# Autodesk Inventor assembly: projectorPanTiltSystem02
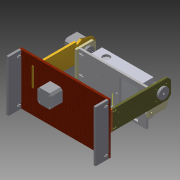
[picture p0: Inventor's stored thumbnail of the model, 180x180]
Saved by Autodesk Inventor 2013 (Build 170138000, 138)
## iProperties
Created: 2014-06-13
Part Number: projectorPanTiltSystem02
Document SubType Name: Assembly
Designer: Byron
Author: Byron
## Documents named in this file (15)
- C:\Users\Nano\Documents\InventorByron\InventorMasterProject\projectorPanTilt02-2014-06-23\projectorPanTilt02\projectorPanTiltSystem02.iam
- C:\Users\Nano\Documents\InventorByron\InventorMasterProject\projectorPanTilt-2014-06-23\projectorPanTilt\stepper42BYGH007.ipt
- C:\Users\Nano\Documents\InventorByron\InventorMasterProject\projectorPanTilt-2014-06-23\projectorPanTilt\aaxaProjector01.ipt
- C:\Users\Nano\Documents\InventorByron\InventorMasterProject\projectorPanTilt02-2014-06-23\projectorPanTilt02\projectorMountingBase.ipt
- C:\Users\Nano\Documents\InventorByron\InventorMasterProject\projectorPanTilt02-2014-06-23\projectorPanTilt02\projectorMountSide.ipt
- C:\Users\Nano\Documents\InventorByron\InventorMasterProject\projectorPanTilt02-2014-06-23\projectorPanTilt02\tiltColumnStepperSide02.ipt
- C:\Users\Nano\Documents\InventorByron\InventorMasterProject\projectorPanTilt02-2014-06-23\projectorPanTilt02\stepperShaftCollar.ipt
- C:\Users\Nano\Documents\InventorByron\InventorMasterProject\projectorPanTilt02-2014-06-23\projectorPanTilt02\tiltStructureCrossBeam.ipt
- C:\Users\Nano\Documents\InventorByron\InventorMasterProject\projectorPanTilt02-2014-06-23\projectorPanTilt02\tiltColumnNonStepperSide02.ipt
- C:\Users\Nano\Documents\InventorByron\InventorMasterProject\projectorPanTilt02-2014-06-23\projectorPanTilt02\panStepperMount.ipt
- C:\Users\Nano\Documents\InventorByron\InventorMasterProject\projectorPanTilt02-2014-06-23\projectorPanTilt02\rotatingSupportShaft.ipt
- C:\Users\Nano\Documents\InventorByron\InventorMasterProject\projectorPanTilt02-2014-06-23\projectorPanTilt02\shaftEndPlate.ipt
- C:\Users\Nano\Documents\InventorByron\InventorMasterProject\projectorPanTilt02-2014-06-23\projectorPanTilt02\cornerBrace.ipt
- C:\Users\Nano\Documents\InventorByron\InventorMasterProject\projectorPanTilt02-2014-06-23\projectorPanTilt02\cornerBrace_MIR.ipt
- C:\Users\Nano\Documents\InventorByron\InventorMasterProject\projectorPanTilt02-2014-06-23\projectorPanTilt02\baseBoxShortSide.ipt
## Components (20 placed, 14 different names)
1. stepper42BYGH007:1 — Mate:13, Flush:10
2. stepper42BYGH007:2 — Flush:7, Mate:2, Mate:3, Mate:7
3. aaxaProjector01:1 — Flush:1, Mate:4
4. projectorMountingBase:1 — Flush:1, Flush:2, Flush:3, Flush:4, Flush:5, Flush:6, Mate:1, Mate:4
5. projectorMountSide:1 — Flush:2, Flush:3, Flush:4, Mate:8, Mate:9, Mate:18
6. projectorMountSide:2 — Flush:5, Flush:6, Mate:1, Mate:5, Mate:6
7. tiltColumnStepperSide02:1 — Flush:7, Mate:2, Mate:3, Angle:1, Mate:9, Mate:24
8. stepperShaftCollar:1 — Mate:7, Mate:8, Mate:18, Mate:23
9. tiltColumnNonStepperSide02:1 — Mate:5, Mate:6, Angle:1, Mate:11, Mate:12, Flush:11, Flush:15, Mate:20, Mate:24
10. tiltStructureCrossBeam:1 — Flush:8, Mate:11, Mate:12, Mate:13, Mate:14, Flush:13, Flush:14
11. panStepperMount:1 — Flush:10, Mate:14, Flush:16, Flush:17, Mate:17, Flush:18, Flush:19
12. rotatingSupportShaft:1 — Flush:11, Flush:12, Mate:16, Mate:21
13. shaftEndPlate:1 — Flush:12, Mate:22
14. shaftEndPlate:2 — Mate:16, Mate:20, Mate:21, Mate:22, Mate:23
15. cornerBrace_MIR:1
16. cornerBrace_MIR:2
17. baseBoxShortSide:1 — Flush:16, Flush:17
18. baseBoxShortSide:2 — Mate:17, Flush:18, Flush:19
19. cornerBrace:1 — Flush:13, Flush:14
20. cornerBrace:2
## Component patterns: (2 elements, first: cornerBrace:1)
## Relationships (40: Mate 21, Flush 18, Angle 1)
- Flush:1: aaxaProjector01:1 ↔ projectorMountingBase:1
- Flush:2: projectorMountingBase:1 ↔ projectorMountSide:1
- Flush:3 (-6.35 mm): projectorMountingBase:1 ↔ projectorMountSide:1
- Flush:4: projectorMountingBase:1 ↔ projectorMountSide:1
- Flush:5: projectorMountingBase:1 ↔ projectorMountSide:2
- Flush:6: projectorMountingBase:1 ↔ projectorMountSide:2
- Mate:1: projectorMountingBase:1 ↔ projectorMountSide:2
- Flush:7: stepper42BYGH007:2 ↔ tiltColumnStepperSide02:1
- Mate:2: stepper42BYGH007:2 ↔ tiltColumnStepperSide02:1
- Mate:3: stepper42BYGH007:2 ↔ tiltColumnStepperSide02:1
- Mate:4: aaxaProjector01:1 ↔ projectorMountingBase:1
- Mate:5 (1.016 mm): projectorMountSide:2 ↔ tiltColumnNonStepperSide02:1
- Mate:6: projectorMountSide:2 ↔ tiltColumnNonStepperSide02:1
- Angle:1 (0 deg): tiltColumnStepperSide02:1 ↔ tiltColumnNonStepperSide02:1
- Mate:7: stepper42BYGH007:2 ↔ stepperShaftCollar:1
- Mate:8: projectorMountSide:1 ↔ stepperShaftCollar:1
- Mate:9 (1.016 mm): projectorMountSide:1 ↔ tiltColumnStepperSide02:1
- Flush:8: tiltStructureCrossBeam:1
- Mate:11: tiltColumnNonStepperSide02:1 ↔ tiltStructureCrossBeam:1
- Mate:12: tiltColumnNonStepperSide02:1 ↔ tiltStructureCrossBeam:1
- Mate:13: stepper42BYGH007:1 ↔ tiltStructureCrossBeam:1
- Flush:10: stepper42BYGH007:1 ↔ panStepperMount:1
- Mate:14: tiltStructureCrossBeam:1 ↔ panStepperMount:1
- Flush:11 (1.016 mm): tiltColumnNonStepperSide02:1 ↔ rotatingSupportShaft:1
- Flush:12: rotatingSupportShaft:1 ↔ shaftEndPlate:1
- Mate:16: rotatingSupportShaft:1 ↔ shaftEndPlate:2
- Flush:13: tiltStructureCrossBeam:1 ↔ cornerBrace:1
- Flush:14: tiltStructureCrossBeam:1 ↔ cornerBrace:1
- Flush:15 (107.95 mm): tiltColumnNonStepperSide02:1
- Flush:16: panStepperMount:1 ↔ baseBoxShortSide:1
- Flush:17: panStepperMount:1 ↔ baseBoxShortSide:1
- Mate:17: panStepperMount:1 ↔ baseBoxShortSide:2
- Flush:18: panStepperMount:1 ↔ baseBoxShortSide:2
- Flush:19: panStepperMount:1 ↔ baseBoxShortSide:2
- Mate:18: projectorMountSide:1 ↔ stepperShaftCollar:1
- Mate:20: tiltColumnNonStepperSide02:1 ↔ shaftEndPlate:2
- Mate:21: rotatingSupportShaft:1 ↔ shaftEndPlate:2
- Mate:22: shaftEndPlate:1 ↔ shaftEndPlate:2
- Mate:23: stepperShaftCollar:1 ↔ shaftEndPlate:2
- Mate:24: tiltColumnStepperSide02:1 ↔ tiltColumnNonStepperSide02:1
